# Autodesk Inventor assembly: Checkpoint
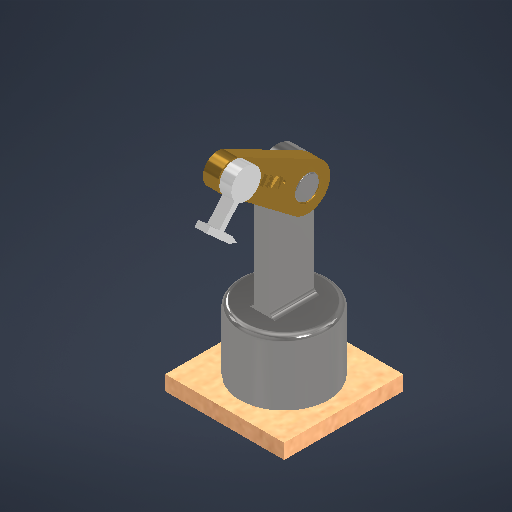
[picture p0: Inventor's stored thumbnail of the model, 512x512]
Saved by Autodesk Inventor 2026.4 (Build 304435000, 435)
## iProperties
Created: 2026-09-01
Part Number: Checkpoint
Document SubType Name: Assembly
Designer: Matheus
Author: Matheus
## Documents named in this file (5)
- C:\Users\win\Downloads\Checkpoint.iam
- C:\Users\win\Downloads\braço do robo.ipt
- C:\Users\win\Downloads\base.ipt
- C:\Users\win\Downloads\solda.ipt
- C:\Users\win\Downloads\Corpo do robo.ipt
## Components (4 placed, 4 different names)
1. braço do robo:1 — Coincidente:1, Alinhado:1, Coincidente:3
2. base:1 — Coincidente:2, Alinhado:2
3. solda:1 — Coincidente:3
4. Corpo do robo:1 — Coincidente:1, Alinhado:1, Coincidente:2, Alinhado:2
## Relationships (5: Mate 3, Flush 2)
- Coincidente:1 [Mate]: braço do robo:1 ↔ Corpo do robo:1
- Alinhado:1 [Flush]: braço do robo:1 ↔ Corpo do robo:1
- Coincidente:2 [Mate]: base:1 ↔ Corpo do robo:1
- Alinhado:2 [Flush]: base:1 ↔ Corpo do robo:1
- Coincidente:3 [Mate]: braço do robo:1 ↔ solda:1
